# Autodesk Inventor assembly: elektromagneet gripper assembly
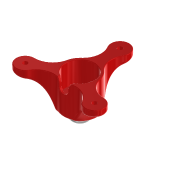
[picture p0: Inventor's stored thumbnail of the model, 180x180]
Saved by Autodesk Inventor 2020.3 (Build 243373000, 373)
## iProperties
Created: 2020-06-22
Part Number: elektromagneet gripper assembly
Document SubType Name: Assembly
Designer: Svend
Author: Svend
## Documents named in this file (3)
- C:\Users\Svend\OneDrive\Documents\GitHub\BeerMinder\3D-model\gripper\elektromagneet gripper assembly.iam
- C:\Users\Svend\OneDrive\Documents\GitHub\BeerMinder\3D-model\3d Prints\elektromagneet.ipt
- C:\Users\Svend\OneDrive\Documents\GitHub\BeerMinder\3D-model\3d Prints\kogel.ipt
## Components (2 placed, 2 different names)
1. elektromagneet:1 — Tangent:1, Mate:1
2. kogel:1 — Tangent:1, Mate:1
## Relationships (2: Tangent 1, Mate 1)
- Tangent:1: elektromagneet:1 ↔ kogel:1
- Mate:1: elektromagneet:1 ↔ kogel:1
